# Autodesk Inventor assembly: Cartesian2_YAssembly
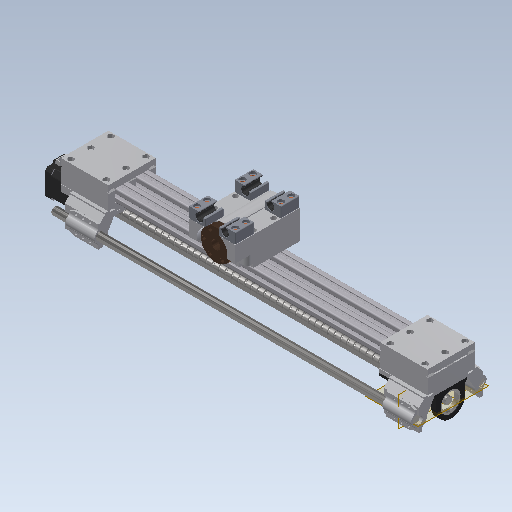
[picture p0: Inventor's stored thumbnail of the model, 512x512]
Saved by Autodesk Inventor 2020 (Build 240168000, 168)
## iProperties
Created: 2020-08-17
Part Number: Cartesian2_YAssembly
Material: Ogólny
Document SubType Name: Assembly
Designer: invin
Mass: 4227.11 g
Surface Area: 5602.37 cm^2
Volume: 1262.4 cm^3
Density: 3.34848 g/cm^3
Author: invin
## Documents named in this file (15)
- D:\KONIECTEGOKOŁCHOZU\MGR\model\Workspaces\Obszar roboczy\Assembly\Y\Y.iam
- D:\KONIECTEGOKOŁCHOZU\MGR\model\Workspaces\Obszar roboczy\Assembly\Y\z2cz.iam
- D:\KONIECTEGOKOŁCHOZU\MGR\model\Workspaces\Obszar roboczy\Assembly\Y\zlozenie_Z.iam
- D:\KONIECTEGOKOŁCHOZU\MGR\model\Workspaces\Obszar roboczy\Assembly\Y\ZY_mount.ipt
- D:\KONIECTEGOKOŁCHOZU\MGR\model\Workspaces\Obszar roboczy\Zawartość\item\item_0037003_Profile_5_20x20_L=564_1.ipt
- D:\KONIECTEGOKOŁCHOZU\MGR\model\Workspaces\Obszar roboczy\Zawartość\Części manipulatora\Cartesian1_12mm_Rod.ipt
- D:\KONIECTEGOKOŁCHOZU\MGR\model\Workspaces\Obszar roboczy\Assembly\Y\Cartesian2_BallBearing_25x37x7.ipt
- D:\KONIECTEGOKOŁCHOZU\MGR\model\Workspaces\Obszar roboczy\Assembly\X\OLD\Cartesian1_X_RodCover.ipt
- D:\KONIECTEGOKOŁCHOZU\MGR\model\Workspaces\Obszar roboczy\Zawartość\nema17\Nema17 Stepper Motor.ipt
- D:\KONIECTEGOKOŁCHOZU\MGR\model\Workspaces\Obszar roboczy\Zawartość\Części manipulatora\Cartesian1_12_12_Clutch.ipt
- D:\KONIECTEGOKOŁCHOZU\MGR\model\Workspaces\Obszar roboczy\Zawartość\Części manipulatora\Cartesian1_BallScrew.ipt
- D:\KONIECTEGOKOŁCHOZU\MGR\model\Workspaces\Obszar roboczy\Assembly\Y\Y_end_cover.ipt
- D:\KONIECTEGOKOŁCHOZU\MGR\model\Workspaces\Obszar roboczy\Assembly\Z\Z_carriage.ipt
- D:\KONIECTEGOKOŁCHOZU\MGR\model\Workspaces\Obszar roboczy\Assembly\Z\Z_nut.ipt
- D:\KONIECTEGOKOŁCHOZU\MGR\model\Workspaces\Obszar roboczy\Zawartość\Igus\WJ200UM_01_10_1.ipt
## Components (23 placed, 14 different names)
1. zlozenie_Z:1 [sub-assembly] — Zestawiający:1, Kąt:1, Zestawiający:6, Zestawiający:7, Zestawiający:9, Zestawiający:10, Zestawiający:13, Zestawiający:32, Zestawiający:33, Zestawiający:34, Zestawiający:35, Zestawiający:36, Zestawiający:37, Zestawiający:44, Kąt:3, Zestawiający:45, Zestawiające:54, Równoległe:6, Równoległe:7, Zestawiające:57, Równoległe:12
2. z2cz:2 [sub-assembly] — Zestawiający:1, Kąt:1, Zestawiający:12, Równoległy:1, Równoległy:2, Zestawiający:24, Zestawiający:25, Zestawiający:26, Zestawiający:27, Zestawiający:28, Zestawiający:29, Zestawiający:30, Zestawiający:31, Zestawiające:50, Równoległe:3, Równoległe:10
3. ZY_mount:1 — Zestawiające:50, Zestawiające:52, Równoległe:3, Zestawiające:53, Równoległe:4, Równoległe:5, Zestawiające:55, Zestawiające:56
4. item_0037003_Profile_5_20x20_L=564_1:1 — Zestawiający:9, Zestawiający:10, Zestawiające:56
5. item_0037003_Profile_5_20x20_L=564_1:2 — Zestawiający:6, Zestawiający:7, Zestawiające:52, Zestawiające:55, Zestawiające:57, Zestawiające:58, Równoległe:11
6. Cartesian1_12mm_Rod:1 — Zestawiający:13, Równoległy:1
7. Cartesian1_12mm_Rod:2 — Zestawiający:12, Równoległy:2
8. Cartesian2_BallBearing_25x37x7:1 — Zestawiający:24, Zestawiający:25
9. Cartesian1_X_RodCover:1 — Zestawiający:26, Zestawiający:27, Zestawiający:28
10. Cartesian1_X_RodCover:2 — Zestawiający:29, Zestawiający:30, Zestawiający:31
11. Cartesian1_X_RodCover:3 — Zestawiający:32, Zestawiający:33, Zestawiający:34
12. Cartesian1_X_RodCover:4 — Zestawiający:35, Zestawiający:36, Zestawiający:37
13. Nema17 Stepper Motor:2 — Zestawiający:44, Kąt:3, Zestawiający:45, Zestawiający:46, Zestawiający:47
14. Cartesian1_12_12_Clutch:1 — Zestawiający:46, Zestawiający:47, Zestawiający:48, Zestawiający:49
15. Cartesian1_BallScrew:1 — Zestawiający:48, Zestawiający:49
16. Y_end_cover:1 — Zestawiające:53, Równoległe:4, Równoległe:5
17. Y_end_cover:2 — Zestawiające:54, Równoległe:6, Równoległe:7, Równoległe:8, Równoległe:9
18. Z_carriage:1 — Zestawiające:58, Równoległe:11, Równoległe:12, Zestawiające:59, Zestawiające:60, Zestawiające:61, Zestawiające:62, Zestawiające:63, Zestawiające:64, Zestawiające:65, Zestawiające:66, Zestawiające:67, Zestawiające:68, Zestawiające:69, Zestawiające:70, Zestawiające:71, Zestawiające:72, Zestawiające:73
19. Z_nut:2 — Zestawiające:59, Zestawiające:60, Zestawiające:61
20. WJ200UM_01_10_1:1 — Zestawiające:62, Zestawiające:63, Zestawiające:64
21. WJ200UM_01_10_1:2 — Zestawiające:65, Zestawiające:66, Zestawiające:67
22. WJ200UM_01_10_1:3 — Zestawiające:68, Zestawiające:69, Zestawiające:70
23. WJ200UM_01_10_1:4 — Zestawiające:71, Zestawiające:72, Zestawiające:73
## Relationships (64: Mate 50, Flush 12, Angle 2)
- Zestawiający:1 [Mate]: zlozenie_Z:1 ↔ z2cz:2
- Kąt:1 [Angle] (0 deg): zlozenie_Z:1 ↔ z2cz:2
- Zestawiający:6 [Mate]: zlozenie_Z:1 ↔ item_0037003_Profile_5_20x20_L=564_1:2
- Zestawiający:7 [Mate]: zlozenie_Z:1 ↔ item_0037003_Profile_5_20x20_L=564_1:2
- Zestawiający:9 [Mate]: zlozenie_Z:1 ↔ item_0037003_Profile_5_20x20_L=564_1:1
- Zestawiający:10 [Mate]: zlozenie_Z:1 ↔ item_0037003_Profile_5_20x20_L=564_1:1
- Zestawiający:12 [Mate]: z2cz:2 ↔ Cartesian1_12mm_Rod:2
- Zestawiający:13 [Mate]: zlozenie_Z:1 ↔ Cartesian1_12mm_Rod:1
- Równoległy:1 [Flush] (4 mm): z2cz:2 ↔ Cartesian1_12mm_Rod:1
- Równoległy:2 [Flush] (4 mm): z2cz:2 ↔ Cartesian1_12mm_Rod:2
- Zestawiający:24 [Mate]: z2cz:2 ↔ Cartesian2_BallBearing_25x37x7:1
- Zestawiający:25 [Mate]: z2cz:2 ↔ Cartesian2_BallBearing_25x37x7:1
- Zestawiający:26 [Mate]: z2cz:2 ↔ Cartesian1_X_RodCover:1
- Zestawiający:27 [Mate]: z2cz:2 ↔ Cartesian1_X_RodCover:1
- Zestawiający:28 [Mate]: z2cz:2 ↔ Cartesian1_X_RodCover:1
- Zestawiający:29 [Mate]: z2cz:2 ↔ Cartesian1_X_RodCover:2
- Zestawiający:30 [Mate]: z2cz:2 ↔ Cartesian1_X_RodCover:2
- Zestawiający:31 [Mate]: z2cz:2 ↔ Cartesian1_X_RodCover:2
- Zestawiający:32 [Mate]: zlozenie_Z:1 ↔ Cartesian1_X_RodCover:3
- Zestawiający:33 [Mate]: zlozenie_Z:1 ↔ Cartesian1_X_RodCover:3
- Zestawiający:34 [Mate]: zlozenie_Z:1 ↔ Cartesian1_X_RodCover:3
- Zestawiający:35 [Mate]: zlozenie_Z:1 ↔ Cartesian1_X_RodCover:4
- Zestawiający:36 [Mate]: zlozenie_Z:1 ↔ Cartesian1_X_RodCover:4
- Zestawiający:37 [Mate]: zlozenie_Z:1 ↔ Cartesian1_X_RodCover:4
- Zestawiający:44 [Mate]: zlozenie_Z:1 ↔ Nema17 Stepper Motor:2
- Kąt:3 [Angle] (0 deg): zlozenie_Z:1 ↔ Nema17 Stepper Motor:2
- Zestawiający:45 [Mate]: zlozenie_Z:1 ↔ Nema17 Stepper Motor:2
- Zestawiający:46 [Mate]: Nema17 Stepper Motor:2 ↔ Cartesian1_12_12_Clutch:1
- Zestawiający:47 [Mate] (6 mm): Nema17 Stepper Motor:2 ↔ Cartesian1_12_12_Clutch:1
- Zestawiający:48 [Mate]: Cartesian1_12_12_Clutch:1 ↔ Cartesian1_BallScrew:1
- Zestawiający:49 [Mate]: Cartesian1_12_12_Clutch:1 ↔ Cartesian1_BallScrew:1
- Zestawiające:50 [Mate]: z2cz:2 ↔ ZY_mount:1
- Zestawiające:52 [Mate]: ZY_mount:1 ↔ item_0037003_Profile_5_20x20_L=564_1:2
- Równoległe:3 [Flush]: z2cz:2 ↔ ZY_mount:1
- Zestawiające:53 [Mate]: ZY_mount:1 ↔ Y_end_cover:1
- Równoległe:4 [Flush]: ZY_mount:1 ↔ Y_end_cover:1
- Równoległe:5 [Flush]: ZY_mount:1 ↔ Y_end_cover:1
- Zestawiające:54 [Mate]: zlozenie_Z:1 ↔ Y_end_cover:2
- Równoległe:6 [Flush]: zlozenie_Z:1 ↔ Y_end_cover:2
- Równoległe:7 [Flush]: zlozenie_Z:1 ↔ Y_end_cover:2
- Równoległe:8 [Flush]: Y_end_cover:2
- Równoległe:9 [Flush]: Y_end_cover:2
- Zestawiające:55 [Mate]: ZY_mount:1 ↔ item_0037003_Profile_5_20x20_L=564_1:2
- Zestawiające:56 [Mate]: ZY_mount:1 ↔ item_0037003_Profile_5_20x20_L=564_1:1
- Zestawiające:57 [Mate]: zlozenie_Z:1 ↔ item_0037003_Profile_5_20x20_L=564_1:2
- Równoległe:10 [Flush]: z2cz:2
- Zestawiające:58 [Mate]: item_0037003_Profile_5_20x20_L=564_1:2 ↔ Z_carriage:1
- Równoległe:11 [Flush] (-9.75 mm): item_0037003_Profile_5_20x20_L=564_1:2 ↔ Z_carriage:1
- Równoległe:12 [Flush] (-216 mm): zlozenie_Z:1 ↔ Z_carriage:1
- Zestawiające:59 [Mate]: Z_carriage:1 ↔ Z_nut:2
- Zestawiające:60 [Mate]: Z_carriage:1 ↔ Z_nut:2
- Zestawiające:61 [Mate]: Z_carriage:1 ↔ Z_nut:2
- Zestawiające:62 [Mate]: Z_carriage:1 ↔ WJ200UM_01_10_1:1
- Zestawiające:63 [Mate]: Z_carriage:1 ↔ WJ200UM_01_10_1:1
- Zestawiające:64 [Mate]: Z_carriage:1 ↔ WJ200UM_01_10_1:1
- Zestawiające:65 [Mate]: Z_carriage:1 ↔ WJ200UM_01_10_1:2
- Zestawiające:66 [Mate]: Z_carriage:1 ↔ WJ200UM_01_10_1:2
- Zestawiające:67 [Mate]: Z_carriage:1 ↔ WJ200UM_01_10_1:2
- Zestawiające:68 [Mate]: Z_carriage:1 ↔ WJ200UM_01_10_1:3
- Zestawiające:69 [Mate]: Z_carriage:1 ↔ WJ200UM_01_10_1:3
- Zestawiające:70 [Mate]: Z_carriage:1 ↔ WJ200UM_01_10_1:3
- Zestawiające:71 [Mate]: Z_carriage:1 ↔ WJ200UM_01_10_1:4
- Zestawiające:72 [Mate]: Z_carriage:1 ↔ WJ200UM_01_10_1:4
- Zestawiające:73 [Mate]: Z_carriage:1 ↔ WJ200UM_01_10_1:4
